# Autodesk Inventor assembly: lcall3
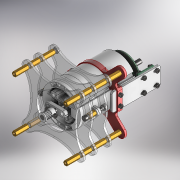
[picture p0: Inventor's stored thumbnail of the model, 180x180]
Saved by Autodesk Inventor 2018 (Build 220112000, 112)
## iProperties
Created: 2018-03-25
Part Number: lcall3
Document SubType Name: Assembly
Designer: mansu
Author: mansu
## Documents named in this file (29)
- F:\OneDrive\Documents\2018 UBC\ELEC 391\Controller\cad\release\lcall3.iam
- F:\OneDrive\Documents\2018 UBC\ELEC 391\Controller\cad\release\YawMotor.iam
- F:\OneDrive\Documents\2018 UBC\ELEC 391\Controller\cad\release\YawMotorPlate.ipt
- F:\OneDrive\Documents\2018 UBC\ELEC 391\Controller\cad\release\Fasteners\StandoffM4x20B.ipt
- F:\OneDrive\Documents\2018 UBC\ELEC 391\Controller\cad\release\Fasteners\StandoffM4x10A.ipt
- F:\OneDrive\Documents\2018 UBC\ELEC 391\Controller\cad\release\Fasteners\StandoffM4x15B.ipt
- F:\OneDrive\Documents\2018 UBC\ELEC 391\Controller\cad\release\EncoderWheelYaw.ipt
- F:\OneDrive\Documents\2018 UBC\ELEC 391\Controller\cad\release\EncoderWheelAdapter.ipt
- C:\Users\mansu\Documents\Inventor\Content Center Files\R2018\en-US\AS 1420\AS 1420 - 1973 - M3 x 8.ipt
- C:\Users\mansu\Documents\Inventor\Content Center Files\R2018\en-US\AS 1474(1)\AS 1474 - M3(1).ipt
- C:\Users\mansu\Documents\Inventor\Content Center Files\R2018\en-US\AS 1420\AS 1420 - 1973 - M3 x 12.ipt
- F:\OneDrive\Documents\2018 UBC\ELEC 391\Controller\cad\release\GT2Yaw.ipt
- C:\Users\mansu\Documents\Inventor\Content Center Files\R2018\en-US\AS 1420\AS 1420 - 1973 - M3 x 14.ipt
- C:\Users\mansu\Documents\Inventor\Content Center Files\R2018\en-US\AS 1420\AS 1420 - 1973 - M4 x 16.ipt
- C:\Users\mansu\Documents\Inventor\Content Center Files\R2018\en-US\AS 1420\AS 1420 - 1973 - M4 x 8.ipt
- F:\OneDrive\Documents\2018 UBC\ELEC 391\Controller\cad\release\EncoderPCBAssembly.iam
- F:\OneDrive\Documents\2018 UBC\ELEC 391\Controller\cad\release\YawBottomPlate.ipt
- F:\OneDrive\Documents\2018 UBC\ELEC 391\Controller\cad\release\Magnet6010.ipt
- C:\Users\mansu\Documents\Inventor\Content Center Files\R2018\en-US\AS 1474(1)\AS 1474 - M4(1).ipt
- F:\OneDrive\Documents\2018 UBC\ELEC 391\Controller\cad\release\Fasteners\StandoffM4x20A.ipt
- F:\OneDrive\Documents\2018 UBC\ELEC 391\Controller\cad\release\YawTopClamp.ipt
- F:\OneDrive\Documents\2018 UBC\ELEC 391\Controller\cad\release\EncoderPCBMount.ipt
- C:\Users\mansu\Documents\Inventor\Content Center Files\R2018\en-US\AS 1420\AS 1420 - 1973 - M3 x 6.ipt
- F:\OneDrive\Documents\2018 UBC\ELEC 391\Controller\cad\release\lcall3\AIP\FEA\cgn2vxe2o.fins
- F:\OneDrive\Documents\2018 UBC\ELEC 391\Controller\cad\release\lcall3\AIP\FEA\cgn2vxe2o.fsat
- F:\OneDrive\Documents\2018 UBC\ELEC 391\Controller\cad\release\lcall3\AIP\FEA\cgn2vxe2o.ftes
- F:\OneDrive\Documents\2018 UBC\ELEC 391\Controller\cad\release\lcall3\AIP\FEA\cgn2vxe2o.fwiz
- F:\OneDrive\Documents\2018 UBC\ELEC 391\Controller\cad\release\lcall3\AIP\FEA\cgn2vxe74.fmsh
- F:\OneDrive\Documents\2018 UBC\ELEC 391\Controller\cad\release\lcall3\AIP\FEA\cgn2vxe75.fres
## Components (58 placed, 22 different names)
1. YawMotor:1 [sub-assembly] — Mate:7, Mate:8, Mate:11, Mate:12, Mate:13, Mate:14, Mate:21, Mate:24, Flush:1, Mate:30, Mate:31, Flush:2, Mate:32, Mate:33, Flush:3, Mate:34, Mate:35, Flush:4, Mate:36, Mate:37, Flush:5, Mate:38, Mate:39, Flush:6, Mate:40, Mate:41, Flush:7
2. YawMotorPlate:1 — Mate:5, Mate:8, Mate:10, Insert:15, Mate:43, Mate:45, Mate:46, Mate:47, Insert:23, Insert:24
3. YawMotorPlate:2 — Mate:6, Mate:7, Insert:3, Insert:4, Mate:11, Insert:5, Insert:6, Insert:7, Insert:8, Insert:9, Insert:10, Insert:11, Insert:12, Insert:16, Insert:17
4. EncoderWheelYaw:1 — Mate:13, Mate:15, Mate:16, Insert:13, Insert:14, Mate:21
5. EncoderWheelAdapter:1 — Mate:14, Mate:15, Mate:16, Mate:18, Mate:20, Mate:22, Tangent:1, Tangent:2
6. GT2Yaw:1 — Mate:24, Flush:1, Mate:25, Tangent:3, Tangent:4
7. AS 1420 - Metric M3 x 14:1 — Mate:25, Tangent:3, Mate:26
8. AS 1474 - Metric M3:4 — Mate:26, Tangent:4
9. AS 1420 - Metric M4 x 16:2 — Insert:15
10. AS 1420 - Metric M4 x 8:1 — Insert:16
11. AS 1420 - Metric M4 x 8:2 — Insert:17
12. EncoderPCBAssembly:1 [sub-assembly] — Tangent:5, Tangent:6, Mate:51, Mate:54, Mate:56, Mate:58, Mate:60, Mate:63, Mate:65, Mate:67, Mate:69
13. YawBottomPlate:1 — Insert:18, Mate:29, Insert:19, Insert:20, Insert:21, Insert:22
14. StandoffM4x20B:11 — Insert:20
15. StandoffM4x20B:12 — Insert:21
16. StandoffM4x20B:13 — Insert:22
17. StandoffM4x20B:14 — Insert:19
18. Magnet6010:1 — Mate:34, Mate:35, Flush:4
19. Magnet6010:2 — Mate:32, Mate:33, Flush:3
20. Magnet6010:3 — Mate:30, Mate:31, Flush:2
21. Magnet6010:4 — Mate:38, Mate:39, Flush:6
22. Magnet6010:5 — Mate:36, Mate:37, Flush:5
23. Magnet6010:6 — Mate:40, Mate:41, Flush:7
24. AS 1474 - Metric M4:1 — Mate:42, Mate:43
25. AS 1474 - Metric M4:2 — Mate:44, Mate:45
26. AS 1420 - Metric M4 x 16:3 — Mate:46, Mate:47
27. StandoffM4x20A:1 — Insert:23, Insert:26
28. StandoffM4x20A:2 — Insert:24, Insert:25
29. YawTopClamp:1 — Insert:25, Insert:26, Mate:48, Mate:49, Mate:50, Mate:52, Mate:53, Insert:27, Mate:70, Mate:71, Mate:73
30. EncoderPCBMount:1 — Mate:48, Mate:49, Mate:50, Tangent:5, Tangent:6, Mate:51, Mate:55, Mate:57, Mate:59, Mate:61
31. AS 1420 - Metric M3 x 6:1 — Mate:52, Mate:53
32. AS 1420 - Metric M3 x 6:2 — Insert:27
33. AS 1420 - Metric M3 x 12:2 — Mate:54, Mate:55, Mate:64
34. AS 1420 - Metric M3 x 12:3 — Mate:56, Mate:57, Mate:62
35. AS 1420 - Metric M3 x 12:4 — Mate:58, Mate:59, Mate:66
36. AS 1420 - Metric M3 x 12:5 — Mate:60, Mate:61, Mate:68
37. AS 1474 - Metric M3:5 — Mate:62, Mate:63
38. AS 1474 - Metric M3:6 — Mate:64, Mate:65
39. AS 1474 - Metric M3:7 — Mate:66, Mate:67
40. AS 1474 - Metric M3:8 — Mate:68, Mate:69
41. AS 1420 - Metric M3 x 8:3 — Mate:70, Mate:71, Mate:72
42. AS 1474 - Metric M3:9 — Mate:72, Mate:73
43. StandoffM4x20B:1 — Insert:4, Mate:10
44. StandoffM4x15B:2 — Insert:3
45. StandoffM4x10A:1 — Insert:5, Mate:12
46. StandoffM4x10A:2 — Insert:6
47. StandoffM4x15B:4 — Insert:7, Mate:29
48. StandoffM4x20B:6 — Insert:8
49. StandoffM4x20B:7 — Insert:12, Mate:42
50. StandoffM4x15B:1 — Insert:11, Insert:18
51. StandoffM4x15B:3 — Insert:9
52. StandoffM4x20B:10 — Insert:10, Mate:44
53. AS 1420 - Metric M3 x 8:1 — Insert:13, Mate:17
54. AS 1420 - Metric M3 x 8:2 — Insert:14, Mate:19
55. AS 1474 - Metric M3:1 — Mate:17, Mate:18
56. AS 1474 - Metric M3:2 — Mate:19, Mate:20
57. AS 1420 - Metric M3 x 12:1 — Mate:22, Tangent:1, Mate:23
58. AS 1474 - Metric M3:3 — Mate:23, Tangent:2
## Relationships (104: Mate 66, Insert 25, Flush 7, Tangent 6)
- Mate:5: YawMotorPlate:1
- Mate:6: YawMotorPlate:2
- Mate:7: YawMotor:1 ↔ YawMotorPlate:2
- Mate:8: YawMotor:1 ↔ YawMotorPlate:1
- Insert:3: YawMotorPlate:2 ↔ StandoffM4x15B:2
- Insert:4: YawMotorPlate:2 ↔ StandoffM4x20B:1
- Mate:10 (0.1 mm): YawMotorPlate:1 ↔ StandoffM4x20B:1
- Mate:11: YawMotor:1 ↔ YawMotorPlate:2
- Insert:5: YawMotorPlate:2 ↔ StandoffM4x10A:1
- Mate:12: YawMotor:1 ↔ StandoffM4x10A:1
- Insert:6: YawMotorPlate:2 ↔ StandoffM4x10A:2
- Insert:7: YawMotorPlate:2 ↔ StandoffM4x15B:4
- Insert:8: YawMotorPlate:2 ↔ StandoffM4x20B:6
- Insert:9: YawMotorPlate:2 ↔ StandoffM4x15B:3
- Insert:10: YawMotorPlate:2 ↔ StandoffM4x20B:10
- Insert:11: YawMotorPlate:2 ↔ StandoffM4x15B:1
- Insert:12: YawMotorPlate:2 ↔ StandoffM4x20B:7
- Mate:13: YawMotor:1 ↔ EncoderWheelYaw:1
- Mate:14: YawMotor:1 ↔ EncoderWheelAdapter:1
- Mate:15: EncoderWheelYaw:1 ↔ EncoderWheelAdapter:1
- Mate:16 (0.1 mm): EncoderWheelYaw:1 ↔ EncoderWheelAdapter:1
- Insert:13: EncoderWheelYaw:1 ↔ AS 1420 - Metric M3 x 8:1
- Insert:14: EncoderWheelYaw:1 ↔ AS 1420 - Metric M3 x 8:2
- Mate:17: AS 1420 - Metric M3 x 8:1 ↔ AS 1474 - Metric M3:1
- Mate:18: EncoderWheelAdapter:1 ↔ AS 1474 - Metric M3:1
- Mate:19: AS 1420 - Metric M3 x 8:2 ↔ AS 1474 - Metric M3:2
- Mate:20: EncoderWheelAdapter:1 ↔ AS 1474 - Metric M3:2
- Mate:21 (10 mm): YawMotor:1 ↔ EncoderWheelYaw:1
- Mate:22: EncoderWheelAdapter:1 ↔ AS 1420 - Metric M3 x 12:1
- Tangent:1 (0.1 mm): EncoderWheelAdapter:1 ↔ AS 1420 - Metric M3 x 12:1
- Mate:23: AS 1420 - Metric M3 x 12:1 ↔ AS 1474 - Metric M3:3
- Tangent:2 (0.1 mm): EncoderWheelAdapter:1 ↔ AS 1474 - Metric M3:3
- Mate:24: YawMotor:1 ↔ GT2Yaw:1
- Flush:1: YawMotor:1 ↔ GT2Yaw:1
- Mate:25: GT2Yaw:1 ↔ AS 1420 - Metric M3 x 14:1
- Tangent:3 (0.1 mm): GT2Yaw:1 ↔ AS 1420 - Metric M3 x 14:1
- Mate:26: AS 1420 - Metric M3 x 14:1 ↔ AS 1474 - Metric M3:4
- Tangent:4 (0.1 mm): GT2Yaw:1 ↔ AS 1474 - Metric M3:4
- Insert:15: YawMotorPlate:1 ↔ AS 1420 - Metric M4 x 16:2
- Insert:16: YawMotorPlate:2 ↔ AS 1420 - Metric M4 x 8:1
- Insert:17: YawMotorPlate:2 ↔ AS 1420 - Metric M4 x 8:2
- Insert:18 (0.1 mm): YawBottomPlate:1 ↔ StandoffM4x15B:1
- Mate:29: YawBottomPlate:1 ↔ StandoffM4x15B:4
- Insert:19: YawBottomPlate:1 ↔ StandoffM4x20B:14
- Insert:20: YawBottomPlate:1 ↔ StandoffM4x20B:11
- Insert:21: YawBottomPlate:1 ↔ StandoffM4x20B:12
- Insert:22: YawBottomPlate:1 ↔ StandoffM4x20B:13
- Mate:30: YawMotor:1 ↔ Magnet6010:3
- Mate:31: YawMotor:1 ↔ Magnet6010:3
- Flush:2 (5 mm): YawMotor:1 ↔ Magnet6010:3
- Mate:32: YawMotor:1 ↔ Magnet6010:2
- Mate:33: YawMotor:1 ↔ Magnet6010:2
- Flush:3 (5 mm): YawMotor:1 ↔ Magnet6010:2
- Mate:34: YawMotor:1 ↔ Magnet6010:1
- Mate:35: YawMotor:1 ↔ Magnet6010:1
- Flush:4 (5 mm): YawMotor:1 ↔ Magnet6010:1
- Mate:36: YawMotor:1 ↔ Magnet6010:5
- Mate:37: YawMotor:1 ↔ Magnet6010:5
- Flush:5 (5 mm): YawMotor:1 ↔ Magnet6010:5
- Mate:38: YawMotor:1 ↔ Magnet6010:4
- Mate:39: YawMotor:1 ↔ Magnet6010:4
- Flush:6 (5 mm): YawMotor:1 ↔ Magnet6010:4
- Mate:40: YawMotor:1 ↔ Magnet6010:6
- Mate:41: YawMotor:1 ↔ Magnet6010:6
- Flush:7 (5 mm): YawMotor:1 ↔ Magnet6010:6
- Mate:42: AS 1474 - Metric M4:1 ↔ StandoffM4x20B:7
- Mate:43: YawMotorPlate:1 ↔ AS 1474 - Metric M4:1
- Mate:44: AS 1474 - Metric M4:2 ↔ StandoffM4x20B:10
- Mate:45: YawMotorPlate:1 ↔ AS 1474 - Metric M4:2
- Mate:46: YawMotorPlate:1 ↔ AS 1420 - Metric M4 x 16:3
- Mate:47: YawMotorPlate:1 ↔ AS 1420 - Metric M4 x 16:3
- Insert:23: YawMotorPlate:1 ↔ StandoffM4x20A:1
- Insert:24: YawMotorPlate:1 ↔ StandoffM4x20A:2
- Insert:25: StandoffM4x20A:2 ↔ YawTopClamp:1
- Insert:26: StandoffM4x20A:1 ↔ YawTopClamp:1
- Mate:48: YawTopClamp:1 ↔ EncoderPCBMount:1
- Mate:49: YawTopClamp:1 ↔ EncoderPCBMount:1
- Mate:50: YawTopClamp:1 ↔ EncoderPCBMount:1
- Tangent:5: EncoderPCBAssembly:1 ↔ EncoderPCBMount:1
- Tangent:6: EncoderPCBAssembly:1 ↔ EncoderPCBMount:1
- Mate:51 (3 mm): EncoderPCBAssembly:1 ↔ EncoderPCBMount:1
- Mate:52: YawTopClamp:1 ↔ AS 1420 - Metric M3 x 6:1
- Mate:53: YawTopClamp:1 ↔ AS 1420 - Metric M3 x 6:1
- Insert:27: YawTopClamp:1 ↔ AS 1420 - Metric M3 x 6:2
- Mate:54: EncoderPCBAssembly:1 ↔ AS 1420 - Metric M3 x 12:2
- Mate:55: EncoderPCBMount:1 ↔ AS 1420 - Metric M3 x 12:2
- Mate:56: EncoderPCBAssembly:1 ↔ AS 1420 - Metric M3 x 12:3
- Mate:57: EncoderPCBMount:1 ↔ AS 1420 - Metric M3 x 12:3
- Mate:58: EncoderPCBAssembly:1 ↔ AS 1420 - Metric M3 x 12:4
- Mate:59: EncoderPCBMount:1 ↔ AS 1420 - Metric M3 x 12:4
- Mate:60: EncoderPCBAssembly:1 ↔ AS 1420 - Metric M3 x 12:5
- Mate:61: EncoderPCBMount:1 ↔ AS 1420 - Metric M3 x 12:5
- Mate:62: AS 1420 - Metric M3 x 12:3 ↔ AS 1474 - Metric M3:5
- Mate:63: EncoderPCBAssembly:1 ↔ AS 1474 - Metric M3:5
- Mate:64: AS 1420 - Metric M3 x 12:2 ↔ AS 1474 - Metric M3:6
- Mate:65: EncoderPCBAssembly:1 ↔ AS 1474 - Metric M3:6
- Mate:66: AS 1420 - Metric M3 x 12:4 ↔ AS 1474 - Metric M3:7
- Mate:67: EncoderPCBAssembly:1 ↔ AS 1474 - Metric M3:7
- Mate:68: AS 1420 - Metric M3 x 12:5 ↔ AS 1474 - Metric M3:8
- Mate:69: EncoderPCBAssembly:1 ↔ AS 1474 - Metric M3:8
- Mate:70: YawTopClamp:1 ↔ AS 1420 - Metric M3 x 8:3
- Mate:71: YawTopClamp:1 ↔ AS 1420 - Metric M3 x 8:3
- Mate:72: AS 1420 - Metric M3 x 8:3 ↔ AS 1474 - Metric M3:9
- Mate:73: YawTopClamp:1 ↔ AS 1474 - Metric M3:9
